# Autodesk Inventor assembly: FullBot
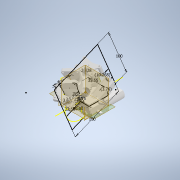
[picture p0: Inventor's stored thumbnail of the model, 180x180]
Saved by Autodesk Inventor 2022 (Build 260153070, 153G)
## iProperties
Created: 2021-11-29
Part Number: FullBot
Document SubType Name: Assembly
Designer: a laptop
Author: a laptop
## Documents named in this file (9)
- C:\Users\a laptop\Desktop\SumoBot\FullBot.iam
- C:\Users\a laptop\Desktop\SumoBot\sumobotENCODER\MotorEncoderAssembly.iam
- C:\Users\a laptop\Desktop\SumoBot\sumobotLIDAR\AssemblyV3.iam
- C:\Users\a laptop\Desktop\SumoBot\sumobotENCODER\REF_PART\TT wheel.ipt
- C:\Users\a laptop\Desktop\SumoBot\sumobotENCODER\MotorEncoderAssembly_MIR.iam
- C:\Users\a laptop\Desktop\SumoBot\Encoderadapter.ipt
- C:\Users\a laptop\Desktop\SumoBot\SumobotSideProfile.ipt
- C:\Users\a laptop\Desktop\SumoBot\REF_PART\2sLIPO.ipt
- C:\Users\a laptop\Desktop\SumoBot\REF_PART\NANO.ipt
## Components (9 placed, 8 different names)
1. MotorEncoderAssembly:1 [sub-assembly] — Angle:1, Mate:7, Mate:8, Angle:6, Flush:3
2. AssemblyV3:1 [sub-assembly] — Angle:1, Mate:12, Mate:11, Flush:4, Mate:13
3. TT wheel:1 — Mate:3, Angle:2, Mate:6, Symmetry:1, Mate:7, Mate:8
4. TT wheel:2 — Mate:3, Angle:2, Mate:6, Tangent:1, Symmetry:1, Mate:9, Mate:10
5. MotorEncoderAssembly_MIR:1 [sub-assembly] — Mate:9, Flush:3, Mate:10, Angle:7
6. Encoderadapter:1 — Flush:4
7. SumobotSideProfile:1 — Mate:11, Mate:13, Angle:8
8. 2sLIPO:1 — Mate:16, Angle:8
9. NANO:1
## Relationships (20: Mate 10, Angle 6, Flush 2, Tangent 1, Symmetry 1)
- Mate:3: TT wheel:1 ↔ TT wheel:2
- Angle:1 (270 deg): MotorEncoderAssembly:1 ↔ AssemblyV3:1
- Angle:2 (0 deg): TT wheel:1 ↔ TT wheel:2
- Mate:6 (-100 mm): TT wheel:1 ↔ TT wheel:2
- Angle:4 (0 deg)
- Tangent:1: TT wheel:2
- Symmetry:1: TT wheel:1 ↔ TT wheel:2
- Mate:12: AssemblyV3:1
- Mate:7: MotorEncoderAssembly:1 ↔ TT wheel:1
- Mate:8: MotorEncoderAssembly:1 ↔ TT wheel:1
- Angle:6 (0 deg): MotorEncoderAssembly:1
- Mate:9: TT wheel:2 ↔ MotorEncoderAssembly_MIR:1
- Flush:3: MotorEncoderAssembly:1 ↔ MotorEncoderAssembly_MIR:1
- Mate:10: TT wheel:2 ↔ MotorEncoderAssembly_MIR:1
- Angle:7 (180 deg): MotorEncoderAssembly_MIR:1
- Mate:11: AssemblyV3:1 ↔ SumobotSideProfile:1
- Flush:4 (1.75 mm): AssemblyV3:1 ↔ Encoderadapter:1
- Mate:13: AssemblyV3:1 ↔ SumobotSideProfile:1
- Mate:16: 2sLIPO:1
- Angle:8 (180 deg): SumobotSideProfile:1 ↔ 2sLIPO:1
